# Autodesk Inventor assembly: Breadboard_Layout
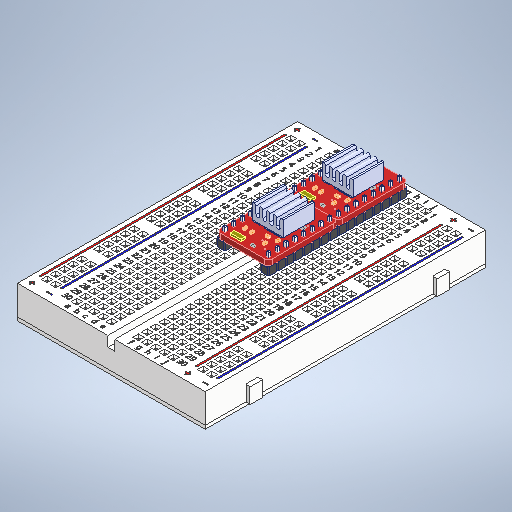
[picture p0: Inventor's stored thumbnail of the model, 512x512]
Saved by Autodesk Inventor 2025.2 (Build 292293000, 293)
## iProperties
Created: 2025-03-19
Part Number: Breadboard_Layout
Document SubType Name: Assembly
Designer: mnguyen6
Author: mnguyen6
## Documents named in this file (3)
- C:\mnguyen\H2A\cad\Misc Electronics\Breadboard_Layout.iam
- C:\mnguyen\H2A\cad\Misc Electronics\Breadboard_half.ipt
- C:\mnguyen\H2A\cad\Misc Electronics\A4988 RED\A4988 RED\A4988 RED.iam
## Components (3 placed, 2 different names)
1. Breadboard_half:1 — Mate:1, Mate:2, Mate:3, Mate:4, Mate:5, Mate:6
2. A4988 RED:1 [sub-assembly] — Mate:1, Mate:2, Mate:3
3. A4988 RED:2 [sub-assembly] — Mate:4, Mate:5, Mate:6
## Relationships (6: Mate 6)
- Mate:1: Breadboard_half:1 ↔ A4988 RED:1
- Mate:2: Breadboard_half:1 ↔ A4988 RED:1
- Mate:3: Breadboard_half:1 ↔ A4988 RED:1
- Mate:4: Breadboard_half:1 ↔ A4988 RED:2
- Mate:5: Breadboard_half:1 ↔ A4988 RED:2
- Mate:6: Breadboard_half:1 ↔ A4988 RED:2
